# Autodesk Inventor assembly: Ensamblaje_Carrito
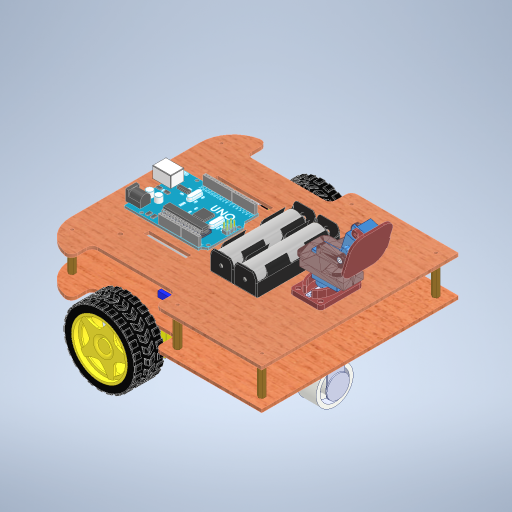
[picture p0: Inventor's stored thumbnail of the model, 512x512]
Saved by Autodesk Inventor 2024 (Build 280153000, 153)
## iProperties
Created: 2025-05-13
Part Number: Ensamblaje_Carrito
Document SubType Name: Assembly
Designer: mario
Author: mario
## Documents named in this file (17)
- C:\Programacion-de-Microcontroladores\Proyecto2\RepositorioProyecto2\Proyecto2_ModelosCAD\Ensamblaje_Carrito.iam
- C:\Programacion-de-Microcontroladores\Proyecto2\RepositorioProyecto2\Proyecto2_ModelosCAD\Importados\Motorreductor\Ensamble de llanta v1\Ensamble de llanta v1.iam
- C:\Users\mario\OneDrive - UVG\Documentos\QUETZAL-2\Base_Carro.ipt
- C:\Users\mario\OneDrive - UVG\Documentos\QUETZAL-2\Soporte_Motorreductor.ipt
- C:\Programacion-de-Microcontroladores\Proyecto2\RepositorioProyecto2\Proyecto2_ModelosCAD\Importados\HolderL.ipt
- C:\Programacion-de-Microcontroladores\Proyecto2\RepositorioProyecto2\Proyecto2_ModelosCAD\Importados\HolderR.ipt
- C:\Programacion-de-Microcontroladores\Proyecto2\RepositorioProyecto2\Proyecto2_ModelosCAD\Importados\Gimbal_2servos\base_nueva.ipt
- C:\Programacion-de-Microcontroladores\Proyecto2\RepositorioProyecto2\Proyecto2_ModelosCAD\Importados\ServoArm\ServoMotor\ServoMotor.ipt
- C:\Programacion-de-Microcontroladores\Proyecto2\RepositorioProyecto2\Proyecto2_ModelosCAD\Importados\ServoArm\Tower pro micro servo SG90 HORN\Tower pro micro servo SG90 HORN.ipt
- C:\Programacion-de-Microcontroladores\Proyecto2\RepositorioProyecto2\Proyecto2_ModelosCAD\Importados\Gimbal_2servos\cabeza_nueva.ipt
- C:\Programacion-de-Microcontroladores\Proyecto2\RepositorioProyecto2\Proyecto2_ModelosCAD\Importados\Portabaterias\18650 Battery Holder v5\18650 Battery Holder v5.ipt
- C:\Programacion-de-Microcontroladores\Proyecto2\RepositorioProyecto2\Proyecto2_ModelosCAD\Importados\L298N\L298N\L298N.ipt
- C:\Programacion-de-Microcontroladores\Proyecto2\RepositorioProyecto2\Proyecto2_ModelosCAD\Importados\Arduino Uno Simplified\Final Assembly\Final Assembly.ipt
- C:\Programacion-de-Microcontroladores\Proyecto2\RepositorioProyecto2\Proyecto2_ModelosCAD\Importados\Gimbal_2servos\Base_Superior.ipt
- C:\Programacion-de-Microcontroladores\Proyecto2\RepositorioProyecto2\Proyecto2_ModelosCAD\Importados\RuedaLoca2\RUEDA LOCA\RUEDA LOCA.ipt
- C:\Programacion-de-Microcontroladores\Proyecto2\RepositorioProyecto2\Proyecto2_ModelosCAD\Importados\Portabaterias_4AA\Batterie nel portabatterie\Batterie nel portabatterie.ipt
- C:\Programacion-de-Microcontroladores\Proyecto2\RepositorioProyecto2\Proyecto2_ModelosCAD\Importados\Gimbal_2servos\Separador M3 x 25 mm.ipt
## Components (25 placed, 16 different names)
1. Ensamble de llanta v1:1 [sub-assembly] — Coincidencia:4, Coincidencia:5, Coincidencia:6
2. Ensamble de llanta v1:2 [sub-assembly] — Coincidencia:10, Coincidencia:11, Coincidencia:12
3. Base_Inferior — Coincidencia:1, Coincidencia:2, Coincidencia:3, Coincidencia:7, Coincidencia:8, Coincidencia:9, Coincidencia:42, Coincidencia:50, Coincidencia:51, Coincidencia:52, Coincidencia:53, Coincidencia:54, Coincidencia:55, Coincidencia:70, Coincidencia:71, Coincidencia:72
4. 18650 Battery Holder v5:1 — Coincidencia:35, Coincidencia:36, Coincidencia:37, Coincidencia:48, Coincidencia:57
5. 18650 Battery Holder v5:2 — Coincidencia:35, Coincidencia:36, Coincidencia:37, Coincidencia:56
6. L298N:1 — Coincidencia:42, Coincidencia:51, Coincidencia:52
7. Arduino Uno — Coincidencia:47, Coincidencia:73, Coincidencia:74, Coincidencia:75
8. Base_Superior:1 — Coincidencia:43, Coincidencia:44, Coincidencia:45, Coincidencia:47, Coincidencia:48, Coincidencia:56, Coincidencia:57, Coincidencia:58, Coincidencia:59, Coincidencia:60, Coincidencia:61, Coincidencia:62, Coincidencia:63, Coincidencia:64, Coincidencia:65, Coincidencia:66, Coincidencia:67, Coincidencia:68, Coincidencia:69, Coincidencia:73, Coincidencia:74, Coincidencia:75
9. RUEDA LOCA:1 — Coincidencia:50
10. Batterie nel portabatterie:1 — Coincidencia:53, Coincidencia:54, Coincidencia:55
11. Separador M3 x 30 mm:1 — Coincidencia:58, Coincidencia:59, Coincidencia:70
12. Separador M3 x 30 mm:2 — Coincidencia:60, Coincidencia:65
13. Separador M3 x 30 mm:3 — Coincidencia:61, Coincidencia:66
14. Separador M3 x 30 mm:4 — Coincidencia:62, Coincidencia:67
15. Separador M3 x 30 mm:5 — Coincidencia:64, Coincidencia:69, Coincidencia:71, Coincidencia:72
16. Separador M3 x 30 mm:6 — Coincidencia:63, Coincidencia:68
17. Soporte_Motorreductor:1 — Coincidencia:1, Coincidencia:2, Coincidencia:3, Coincidencia:4, Coincidencia:5, Coincidencia:6
18. Soporte_Motorreductor:2 — Coincidencia:7, Coincidencia:8, Coincidencia:9, Coincidencia:10, Coincidencia:11, Coincidencia:12
19. HolderL:1 — Coincidencia:22, Coincidencia:23, Coincidencia:24, Coincidencia:32
20. HolderR:1 — Coincidencia:25, Coincidencia:26, Coincidencia:27, Coincidencia:28
21. base_nueva:1 — Coincidencia:18, Coincidencia:19, Coincidencia:43, Coincidencia:44, Coincidencia:45, Coincidencia:46
22. ServoMotor:1 — Coincidencia:14, Coincidencia:15, Coincidencia:22, Coincidencia:23, Coincidencia:24, Coincidencia:25, Coincidencia:26, Coincidencia:27
23. Tower pro micro servo SG90 HORN:1 — Coincidencia:14, Coincidencia:15, Coincidencia:18, Coincidencia:19, Coincidencia:46
24. ServoMotor:2 — Coincidencia:28, Coincidencia:29, Coincidencia:30, Coincidencia:31
25. cabeza_nueva:1 — Coincidencia:29, Coincidencia:30, Coincidencia:31, Coincidencia:32
## Relationships (63: Mate 63)
- Coincidencia:1 [Mate]: Base_Inferior ↔ Soporte_Motorreductor:1
- Coincidencia:2 [Mate]: Base_Inferior ↔ Soporte_Motorreductor:1
- Coincidencia:3 [Mate]: Base_Inferior ↔ Soporte_Motorreductor:1
- Coincidencia:4 [Mate]: Ensamble de llanta v1:1 ↔ Soporte_Motorreductor:1
- Coincidencia:5 [Mate]: Ensamble de llanta v1:1 ↔ Soporte_Motorreductor:1
- Coincidencia:6 [Mate]: Ensamble de llanta v1:1 ↔ Soporte_Motorreductor:1
- Coincidencia:7 [Mate]: Base_Inferior ↔ Soporte_Motorreductor:2
- Coincidencia:8 [Mate]: Base_Inferior ↔ Soporte_Motorreductor:2
- Coincidencia:9 [Mate]: Base_Inferior ↔ Soporte_Motorreductor:2
- Coincidencia:10 [Mate]: Ensamble de llanta v1:2 ↔ Soporte_Motorreductor:2
- Coincidencia:11 [Mate]: Ensamble de llanta v1:2 ↔ Soporte_Motorreductor:2
- Coincidencia:12 [Mate]: Ensamble de llanta v1:2 ↔ Soporte_Motorreductor:2
- Coincidencia:14 [Mate]: ServoMotor:1 ↔ Tower pro micro servo SG90 HORN:1
- Coincidencia:15 [Mate]: ServoMotor:1 ↔ Tower pro micro servo SG90 HORN:1
- Coincidencia:18 [Mate]: base_nueva:1 ↔ Tower pro micro servo SG90 HORN:1
- Coincidencia:19 [Mate]: base_nueva:1 ↔ Tower pro micro servo SG90 HORN:1
- Coincidencia:22 [Mate]: HolderL:1 ↔ ServoMotor:1
- Coincidencia:23 [Mate]: HolderL:1 ↔ ServoMotor:1
- Coincidencia:24 [Mate]: HolderL:1 ↔ ServoMotor:1
- Coincidencia:25 [Mate]: HolderR:1 ↔ ServoMotor:1
- Coincidencia:26 [Mate]: HolderR:1 ↔ ServoMotor:1
- Coincidencia:27 [Mate]: HolderR:1 ↔ ServoMotor:1
- Coincidencia:28 [Mate]: HolderR:1 ↔ ServoMotor:2
- Coincidencia:29 [Mate]: ServoMotor:2 ↔ cabeza_nueva:1
- Coincidencia:30 [Mate]: ServoMotor:2 ↔ cabeza_nueva:1
- Coincidencia:31 [Mate]: ServoMotor:2 ↔ cabeza_nueva:1
- Coincidencia:32 [Mate]: HolderL:1 ↔ cabeza_nueva:1
- Coincidencia:35 [Mate]: 18650 Battery Holder v5:1 ↔ 18650 Battery Holder v5:2
- Coincidencia:36 [Mate]: 18650 Battery Holder v5:1 ↔ 18650 Battery Holder v5:2
- Coincidencia:37 [Mate]: 18650 Battery Holder v5:1 ↔ 18650 Battery Holder v5:2
- Coincidencia:42 [Mate]: Base_Inferior ↔ L298N:1
- Coincidencia:43 [Mate]: Base_Superior:1 ↔ base_nueva:1
- Coincidencia:44 [Mate]: Base_Superior:1 ↔ base_nueva:1
- Coincidencia:45 [Mate]: Base_Superior:1 ↔ base_nueva:1
- Coincidencia:46 [Mate]: base_nueva:1 ↔ Tower pro micro servo SG90 HORN:1
- Coincidencia:47 [Mate]: Arduino Uno ↔ Base_Superior:1
- Coincidencia:48 [Mate]: 18650 Battery Holder v5:1 ↔ Base_Superior:1
- Coincidencia:50 [Mate]: Base_Inferior ↔ RUEDA LOCA:1
- Coincidencia:51 [Mate]: Base_Inferior ↔ L298N:1
- Coincidencia:52 [Mate]: Base_Inferior ↔ L298N:1
- Coincidencia:53 [Mate]: Base_Inferior ↔ Batterie nel portabatterie:1
- Coincidencia:54 [Mate] (72 mm): Base_Inferior ↔ Batterie nel portabatterie:1
- Coincidencia:55 [Mate] (34.685 mm): Base_Inferior ↔ Batterie nel portabatterie:1
- Coincidencia:56 [Mate]: 18650 Battery Holder v5:2 ↔ Base_Superior:1
- Coincidencia:57 [Mate]: 18650 Battery Holder v5:1 ↔ Base_Superior:1
- Coincidencia:58 [Mate]: Base_Superior:1 ↔ Separador M3 x 30 mm:1
- Coincidencia:59 [Mate]: Base_Superior:1 ↔ Separador M3 x 30 mm:1
- Coincidencia:60 [Mate]: Base_Superior:1 ↔ Separador M3 x 30 mm:2
- Coincidencia:61 [Mate]: Base_Superior:1 ↔ Separador M3 x 30 mm:3
- Coincidencia:62 [Mate]: Base_Superior:1 ↔ Separador M3 x 30 mm:4
- Coincidencia:63 [Mate]: Base_Superior:1 ↔ Separador M3 x 30 mm:6
- Coincidencia:64 [Mate]: Base_Superior:1 ↔ Separador M3 x 30 mm:5
- Coincidencia:65 [Mate]: Base_Superior:1 ↔ Separador M3 x 30 mm:2
- Coincidencia:66 [Mate]: Base_Superior:1 ↔ Separador M3 x 30 mm:3
- Coincidencia:67 [Mate]: Base_Superior:1 ↔ Separador M3 x 30 mm:4
- Coincidencia:68 [Mate]: Base_Superior:1 ↔ Separador M3 x 30 mm:6
- Coincidencia:69 [Mate]: Base_Superior:1 ↔ Separador M3 x 30 mm:5
- Coincidencia:70 [Mate]: Base_Inferior ↔ Separador M3 x 30 mm:1
- Coincidencia:71 [Mate]: Base_Inferior ↔ Separador M3 x 30 mm:5
- Coincidencia:72 [Mate]: Base_Inferior ↔ Separador M3 x 30 mm:5
- Coincidencia:73 [Mate]: Arduino Uno ↔ Base_Superior:1
- Coincidencia:74 [Mate]: Arduino Uno ↔ Base_Superior:1
- Coincidencia:75 [Mate]: Arduino Uno ↔ Base_Superior:1
